# Autodesk Inventor assembly: Trunk
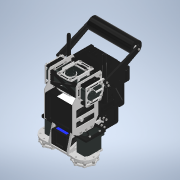
[picture p0: Inventor's stored thumbnail of the model, 180x180]
Saved by Autodesk Inventor 2020.4 (Build 244396000, 396)
## iProperties
Created: 2021-09-10
Part Number: Trunk
Document SubType Name: Assembly
Designer: Masato
Mass: 1663.74 g
Surface Area: 5902.56 cm^2
Volume: 962.647 cm^3
Density: 1.72829 g/cm^3
Author: Masato
## Documents named in this file (38)
- C:\Users\Masato\Documents\Inventor\CIT Brains_Inventor\OpenPlatform_ver3_0\UpperBody\Trunk\Trunk.iam
- C:\Users\Masato\Documents\Inventor\CIT Brains_Inventor\OpenPlatform_ver3_0\UpperBody\Trunk\Trunk_horizontal_frame_03.ipt
- C:\Users\Masato\Documents\Inventor\CIT Brains_Inventor\OpenPlatform_ver3_0\UpperBody\Trunk\Trunk_horizontal_frame_04.ipt
- C:\Users\Masato\Documents\Inventor\CIT Brains_Inventor\OpenPlatform_ver3_0\UpperBody\Trunk\Trunk_horizontal_frame_05.ipt
- C:\Users\Masato\Documents\Inventor\CIT Brains_Inventor\OpenPlatform_ver3_0\UpperBody\Trunk\Trunk_vertical_frame_02.ipt
- C:\Users\Masato\Documents\Inventor\CIT Brains_Inventor\OpenPlatform_ver3_0\UpperBody\Trunk\Trunk_vertical_frame_03.ipt
- C:\Users\Masato\Documents\Inventor\CIT Brains_Inventor\OpenPlatform_ver3_0\UpperBody\Trunk\Trunk_vertical_frame_04.ipt
- C:\Users\Masato\Documents\Inventor\CIT Brains_Inventor\OpenPlatform_ver3_0\UpperBody\Trunk\Trunk_vertical_frame_05.ipt
- C:\Users\Masato\Documents\Inventor\CIT Brains_Inventor\OpenPlatform_ver3_0\UpperBody\Trunk\Trunk_vertical_frame_06.ipt
- C:\Users\Masato\Documents\Inventor\CIT Brains_Inventor\OpenPlatform_ver3_0\Ready_Made\B3M11xx.ipt
- C:\Users\Masato\Documents\Inventor\CIT Brains_Inventor\OpenPlatform_ver3_0\Ready_Made\S3-07-3W.ipt
- C:\Users\Masato\Documents\Inventor\CIT Brains_Inventor\OpenPlatform_ver3_0\Ready_Made\ASU-375H.ipt
- C:\Users\Masato\Documents\Inventor\CIT Brains_Inventor\OpenPlatform_ver3_0\Ready_Made\MSU-306-03.ipt
- C:\Users\Masato\Documents\Inventor\CIT Brains_Inventor\OpenPlatform_ver3_0\Ready_Made\SLSBF7-130-M3-N3.ipt
- C:\Users\Masato\Documents\Inventor\CIT Brains_Inventor\OpenPlatform_ver3_0\Ready_Made\B3M10xx.ipt
- C:\Users\Masato\Documents\Inventor\CIT Brains_Inventor\OpenPlatform_ver3_0\Ready_Made\SGB-100.ipt
- C:\Users\Masato\Documents\Inventor\CIT Brains_Inventor\OpenPlatform_ver3_0\UpperBody\Cockpit\Cockpit.iam
- C:\Users\Masato\Documents\Inventor\CIT Brains_Inventor\OpenPlatform_ver3_0\UpperBody\Trunk\Trunk_vertical_frame_04_MIR.ipt
- C:\Users\Masato\Documents\Inventor\CIT Brains_Inventor\OpenPlatform_ver3_0\UpperBody\Trunk\Trunk_vertical_frame_01.ipt
- C:\Users\Masato\Documents\Inventor\CIT Brains_Inventor\OpenPlatform_ver3_0\UpperBody\Trunk\Trunk_vertical_frame_01_MIR.ipt
- C:\Users\Masato\Documents\Inventor\CIT Brains_Inventor\OpenPlatform_ver3_0\Ready_Made\Screw\SPNFL-BRN-M3-6.ipt
- C:\Users\Masato\Documents\Inventor\CIT Brains_Inventor\OpenPlatform_ver3_0\Ready_Made\Screw\M2_6-15.ipt
- C:\Users\Masato\Documents\Inventor\CIT Brains_Inventor\OpenPlatform_ver3_0\Ready_Made\Screw\M3-8.ipt
- C:\Users\Masato\Documents\Inventor\CIT Brains_Inventor\OpenPlatform_ver3_0\Ready_Made\Screw\M3-6.ipt
- C:\Users\Masato\Documents\Inventor\CIT Brains_Inventor\OpenPlatform_ver3_0\Ready_Made\Screw\M2_6-20.ipt
- C:\Users\Masato\Documents\Inventor\CIT Brains_Inventor\OpenPlatform_ver3_0\UpperBody\Trunk\Outer_support_stand.ipt
- C:\Users\Masato\Documents\Inventor\CIT Brains_Inventor\OpenPlatform_ver3_0\Ready_Made\BRU-307S.ipt
- C:\Users\Masato\Documents\Inventor\CIT Brains_Inventor\OpenPlatform_ver3_0\UpperBody\Trunk\Outer_flange.ipt
- C:\Users\Masato\Documents\Inventor\CIT Brains_Inventor\OpenPlatform_ver3_0\UpperBody\Trunk\Inner_flange.ipt
- C:\Users\Masato\Documents\Inventor\CIT Brains_Inventor\OpenPlatform_ver3_0\Ready_Made\CRBA02508WWC8P5\CRBA02508WWC8P5.ipt
- C:\Users\Masato\Documents\Inventor\CIT Brains_Inventor\OpenPlatform_ver3_0\UpperBody\Trunk\Inner_support_stand.ipt
- C:\Users\Masato\Documents\Inventor\CIT Brains_Inventor\OpenPlatform_ver3_0\UpperBody\Trunk\Trunk_horizontal_frame_01.ipt
- C:\Users\Masato\Documents\Inventor\CIT Brains_Inventor\OpenPlatform_ver3_0\Ready_Made\SF319.ipt
- C:\Users\Masato\Documents\Inventor\CIT Brains_Inventor\OpenPlatform_ver3_0\Ready_Made\BRU-2609S.ipt
- C:\Users\Masato\Documents\Inventor\CIT Brains_Inventor\OpenPlatform_ver3_0\Ready_Made\Screw\M2_6-8.ipt
- C:\Users\Masato\Documents\Inventor\CIT Brains_Inventor\OpenPlatform_ver3_0\UpperBody\Trunk\Trunk_horizontal_frame_02.ipt
- C:\Users\Masato\Documents\Inventor\CIT Brains_Inventor\OpenPlatform_ver3_0\Ready_Made\UUW-0312-10BH.ipt
- C:\Users\Masato\Documents\Inventor\CIT Brains_Inventor\OpenPlatform_ver3_0\Ready_Made\Screw\M2_6-6.ipt
## Components (229 placed, 37 different names)
1. Trunk_horizontal_frame_03:1 — 挿入:172, 挿入:173, 挿入:174, 挿入:175, 挿入:177, 挿入:179, 挿入:255, 挿入:256, 挿入:261, 挿入:262, 挿入:347, 挿入:348, 挿入:463, 挿入:464
2. Trunk_horizontal_frame_03:2 — 挿入:181, 挿入:182, 挿入:184, 挿入:185, 挿入:186, 挿入:187, 挿入:257, 挿入:258, 挿入:337, 挿入:338, 挿入:465, 挿入:466
3. Trunk_horizontal_frame_04:1 — 挿入:115, 挿入:116, 挿入:117, 挿入:118, 挿入:172, 挿入:173, 挿入:181, 挿入:182
4. Trunk_horizontal_frame_04:2 — 挿入:154, 挿入:155, 挿入:156, 挿入:157, 挿入:174, 挿入:175, 挿入:185, 挿入:187
5. Trunk_horizontal_frame_05:1 — 挿入:111, 挿入:112, 挿入:126, 挿入:127
6. Trunk_horizontal_frame_05:2 — 挿入:162, 挿入:163, 挿入:164, 挿入:165
7. Trunk_horizontal_frame_05:3 — 挿入:229, 挿入:230, 挿入:231, 挿入:232
8. Trunk_horizontal_frame_05:4 — 挿入:166, 挿入:167, 挿入:168, 挿入:169
9. Trunk_vertical_frame_01:1 — 角度:35, 角度:36, 挿入:200, 挿入:201, 挿入:420, 挿入:421, 挿入:426, 挿入:501, 挿入:502
10. Trunk_vertical_frame_01_MIR:1 — 角度:37, 角度:38, 挿入:202, 挿入:203, メイト:23, メイト:24, メイト:25, 挿入:418, 挿入:419, 挿入:499, 挿入:500
11. Trunk_vertical_frame_02:1 — フラッシュ:16, メイト:17, フラッシュ:18, フラッシュ:20, フラッシュ:21, メイト:22
12. Trunk_vertical_frame_02:2 — フラッシュ:16, メイト:17, フラッシュ:18, メイト:19
13. Trunk_vertical_frame_02:3 — フラッシュ:15, メイト:18, フラッシュ:17, フラッシュ:19, フラッシュ:20, フラッシュ:21, メイト:21, メイト:20
14. Trunk_vertical_frame_02:4 — フラッシュ:15, メイト:18, フラッシュ:17, メイト:25
15. Trunk_vertical_frame_03:1 — 挿入:101, 挿入:102, 挿入:103, 挿入:111, 挿入:112, 挿入:115, 挿入:116, 挿入:156, 挿入:157, 挿入:164, 挿入:165, フラッシュ:19, メイト:21, 挿入:208, 挿入:226, 挿入:245, 挿入:246, 挿入:247, 挿入:251, 挿入:252, 挿入:327, 挿入:328, 挿入:329, 挿入:330, 挿入:349, 挿入:350
16. Trunk_vertical_frame_03:2 — 挿入:104, 挿入:105, 挿入:106, 挿入:117, 挿入:118, 挿入:154, 挿入:155, 挿入:168, 挿入:169, メイト:22, 挿入:227, 挿入:229, 挿入:230, 挿入:248, 挿入:249, 挿入:250, 挿入:253, 挿入:254, 挿入:331, 挿入:332, 挿入:333, 挿入:334, 挿入:351, 挿入:352
17. Trunk_vertical_frame_04:1 — 挿入:142, 挿入:143, 挿入:144, 挿入:145, 角度:31, 角度:32, 挿入:150, 挿入:151, 挿入:166, 挿入:167, 挿入:231, 挿入:232, 挿入:315, 挿入:316, 挿入:317, 挿入:318, 挿入:323, 挿入:324, 挿入:325, 挿入:326
18. Trunk_vertical_frame_04_MIR:1 — 挿入:124, 挿入:125, 挿入:126, 挿入:127, 挿入:128, 挿入:129, 挿入:136, 挿入:137, 角度:33, 角度:34, 挿入:152, 挿入:153, 挿入:162, 挿入:163, 挿入:311, 挿入:312, 挿入:313, 挿入:314, 挿入:319, 挿入:320, 挿入:321, 挿入:322
19. Trunk_vertical_frame_05:1 — 角度:17, 角度:18, 挿入:75, 挿入:76, 角度:21, 挿入:79, メイト:16, 挿入:263, 挿入:264, 挿入:267
20. Trunk_vertical_frame_05:2 — 角度:19, 挿入:77, 挿入:78, 角度:20, 角度:22, 挿入:80, 挿入:265, 挿入:266, 挿入:268
21. Trunk_vertical_frame_06:1 — 挿入:467, 挿入:468, 挿入:469, 挿入:470, 挿入:471, 挿入:472, 挿入:473, 挿入:474
22. Trunk_vertical_frame_06:2 — 挿入:475, 挿入:476, 挿入:477, 挿入:478, 挿入:479, 挿入:480, 挿入:481, 挿入:482
23. B3M11xx:1 — 角度:39, 挿入:391, 挿入:392, 挿入:422, 挿入:423, 挿入:424, 挿入:425, 挿入:483, 挿入:486
24. B3M11xx:2 — 挿入:427, 挿入:428, 挿入:429, 挿入:484, 挿入:485, 挿入:529
25. B3M11xx:3 — 挿入:177, 挿入:179, 挿入:184, 挿入:186
26. B3M10xx:4 — 挿入:124, 挿入:125, 挿入:128, 挿入:129, 挿入:475, 挿入:476, 挿入:477, 挿入:478
27. B3M10xx:5 — 挿入:142, 挿入:143, 挿入:144, 挿入:145, 挿入:467, 挿入:468, 挿入:469, 挿入:470
28. S3-07-3W:1 — 角度:37, 挿入:202
29. S3-07-3W:2 — 角度:38, 挿入:203
30. S3-07-3W:3 — 角度:36, 挿入:201
31. S3-07-3W:4 — 角度:35, 挿入:200
32. S3-07-3W:5 — 角度:33, 挿入:152
33. S3-07-3W:6 — 角度:34, 挿入:153
34. S3-07-3W:7 — 角度:31, 挿入:150
35. S3-07-3W:8 — 角度:32, 挿入:151
36. ASU-375H:1 — フラッシュ:9, フラッシュ:10, フラッシュ:11, フラッシュ:12, 挿入:101, 挿入:104, メイト:19, メイト:20, メイト:23, メイト:24
37. ASU-375H:2 — フラッシュ:9, フラッシュ:11, 挿入:102, 挿入:105
38. ASU-375H:3 — フラッシュ:10, フラッシュ:12, 挿入:103, 挿入:106
39. MSU-306-03:5 — 角度:17, 挿入:75, 挿入:136
40. MSU-306-03:6 — 角度:18, 挿入:76, 挿入:137
41. MSU-306-03:11 — 角度:19, 挿入:77
42. MSU-306-03:12 — 挿入:78, 角度:20
43. SLSBF7-130-M3-N3:1 — 角度:21, 角度:22, 挿入:79, 挿入:80, メイト:15
44. SGB-100:1 — メイト:15, メイト:16
45. Cockpit:1 [sub-assembly] — 挿入:208, 角度:39
46. SPNFL-BRN-M3-6:1 — 挿入:226
47. SPNFL-BRN-M3-6:2 — 挿入:227
48. M3-8:5 — 挿入:245
49. M3-8:6 — 挿入:246
50. M3-8:7 — 挿入:247
51. M3-8:8 — 挿入:248
52. M3-8:9 — 挿入:249
53. M3-8:10 — 挿入:250
54. M3-6:1 — 挿入:251
55. M3-6:2 — 挿入:252
56. M3-6:3 — 挿入:254
57. M3-6:4 — 挿入:253
58. M3-6:5 — 挿入:256
59. M3-6:6 — 挿入:255
60. M3-6:7 — 挿入:258
61. M3-6:8 — 挿入:257
62. M2_6-15:9 — 挿入:464
63. M2_6-15:10 — 挿入:463
64. M2_6-15:11 — 挿入:261
65. M2_6-15:12 — 挿入:262
66. M3-6:9 — 挿入:263
67. M3-6:10 — 挿入:264
68. M3-6:11 — 挿入:266
69. M3-6:12 — 挿入:265
70. M3-8:11 — 挿入:267
71. M3-8:12 — 挿入:268
72. M2_6-20:1 — 挿入:489
73. M2_6-20:2 — 挿入:490
74. M2_6-20:3 — 挿入:487
75. M2_6-20:4 — 挿入:488
76. M2_6-15:13 — 挿入:311
77. M2_6-15:14 — 挿入:312
78. M2_6-15:15 — 挿入:313
79. M2_6-15:16 — 挿入:314
80. M2_6-15:17 — 挿入:315
81. M2_6-15:18 — 挿入:316
82. M2_6-15:19 — 挿入:317
83. M2_6-15:20 — 挿入:318
84. M3-6:13 — 挿入:319
85. M3-6:14 — 挿入:320
86. M3-6:15 — 挿入:321
87. M3-6:16 — 挿入:322
88. M3-6:17 — 挿入:323
89. M3-6:18 — 挿入:324
90. M3-6:19 — 挿入:325
91. M3-6:20 — 挿入:326
92. M3-6:21 — 挿入:327
93. M3-6:22 — 挿入:328
94. M3-6:23 — 挿入:329
95. M3-6:24 — 挿入:330
96. M3-6:25 — 挿入:331
97. M3-6:26 — 挿入:332
98. M3-6:27 — 挿入:333
99. M3-6:28 — 挿入:334
100. M2_6-20:9 — 挿入:465
101. M2_6-20:10 — 挿入:466
102. M2_6-20:11 — 挿入:337
103. M2_6-20:12 — 挿入:338
104. M2_6-20:13 — 挿入:479
105. M2_6-20:14 — 挿入:482
106. M2_6-20:15 — 挿入:481
107. M2_6-20:16 — 挿入:480
108. M2_6-20:17 — 挿入:474
109. M2_6-20:18 — 挿入:472
110. M2_6-20:19 — 挿入:473
111. M2_6-20:20 — 挿入:471
112. M3-6:29 — 挿入:347
113. M3-6:30 — 挿入:348
114. M3-6:31 — 挿入:349
115. M3-6:32 — 挿入:350
116. M3-6:33 — 挿入:351
117. M3-6:34 — 挿入:352
118. Outer_support_stand:1 — 挿入:371, 挿入:372, 挿入:373, 挿入:374, 挿入:375, 挿入:376, 挿入:377, 挿入:378, 挿入:397, 挿入:438, 挿入:439
119. BRU-307S:1 — 挿入:371, 挿入:404
120. BRU-307S:2 — 挿入:372
121. BRU-307S:3 — 挿入:373
122. BRU-307S:4 — 挿入:374
123. BRU-307S:5 — 挿入:375, 挿入:405
124. BRU-307S:6 — 挿入:376
125. BRU-307S:7 — 挿入:377
126. BRU-307S:8 — 挿入:378
127. Inner_flange:1 — 挿入:391, 挿入:392, 挿入:452, 挿入:453, 挿入:454, 挿入:455
128. CRBA02508WWC8P5:1 — 挿入:397
129. Inner_support_stand:1 — 角度:40, 挿入:398, 角度:41, 挿入:399, 角度:42, 挿入:400, 角度:43, 挿入:401, 挿入:456, 挿入:457, 挿入:458, 挿入:459, 挿入:460, 挿入:461
130. S3-07-3W:9 — 角度:40, 挿入:398
131. S3-07-3W:10 — 角度:41, 挿入:399
132. S3-07-3W:11 — 角度:42, 挿入:400
133. S3-07-3W:12 — 角度:43, 挿入:401
134. Outer_flange:1 — 挿入:404, 挿入:405, 挿入:406, 挿入:407, 挿入:408, 挿入:409, 挿入:410, 挿入:411, 挿入:412, 挿入:413
135. M3-6:35 — 挿入:406
136. M3-6:36 — 挿入:407
137. M3-6:37 — 挿入:408
138. M3-6:38 — 挿入:409
139. M3-6:39 — 挿入:410
140. M3-6:40 — 挿入:411
141. M3-6:41 — 挿入:412
142. M3-6:42 — 挿入:413
143. Trunk_horizontal_frame_01:1 — 挿入:418, 挿入:419, 挿入:420, 挿入:421, 挿入:422, 挿入:423, 挿入:424, 挿入:425, 挿入:426, 挿入:427, 挿入:428, 挿入:429, 挿入:430, 挿入:431, 挿入:432, 挿入:433, 挿入:434, 挿入:435, 挿入:436, 挿入:440, 挿入:441, 挿入:442, 挿入:443, 挿入:444, 挿入:445, 挿入:446, 挿入:447, 挿入:448, 挿入:449, 挿入:450, 挿入:451, フラッシュ:22, 挿入:462, 挿入:511, 挿入:512, 挿入:513, 挿入:514, 挿入:515, 挿入:516, 挿入:517, 挿入:518
144. SF319:1 — 挿入:430
145. SF319:2 — 挿入:431
146. SF319:3 — 挿入:432
147. SF319:4 — 挿入:433, 挿入:439
148. SF319:5 — 挿入:434
149. SF319:6 — 挿入:435
150. SF319:7 — 挿入:436, 挿入:438
151. SF319:8 — 挿入:462
152. M2_6-15:21 — 挿入:441
153. M2_6-15:22 — 挿入:440
154. M2_6-15:23 — 挿入:442
155. M2_6-15:24 — 挿入:443
156. M2_6-15:25 — 挿入:444
157. M2_6-15:26 — 挿入:445
158. M2_6-15:27 — 挿入:446
159. M2_6-15:28 — 挿入:447
160. M3-8:13 — 挿入:448
161. M3-8:14 — 挿入:449
162. M3-8:15 — 挿入:450
163. M3-8:16 — 挿入:451
164. BRU-2609S:1 — 挿入:455, 挿入:457
165. BRU-2609S:2 — 挿入:454
166. BRU-2609S:3 — 挿入:453
167. BRU-2609S:4 — 挿入:452, 挿入:456
168. M2_6-8:1 — 挿入:458
169. M2_6-8:2 — 挿入:459
170. M2_6-8:3 — 挿入:460
171. M2_6-8:4 — 挿入:461
172. Trunk_horizontal_frame_02:1 — 挿入:483, 挿入:484, 挿入:485, 挿入:486, 挿入:487, 挿入:488, 挿入:489, 挿入:490
173. BRU-307S:9 — 挿入:497, 挿入:503
174. BRU-307S:10 — 挿入:498, 挿入:504
175. BRU-307S:11 — 挿入:496, 挿入:506
176. BRU-307S:12 — 挿入:495, 挿入:505
177. UUW-0312-10BH:1 — 挿入:495, 挿入:507
178. UUW-0312-10BH:2 — 挿入:496, 挿入:508
179. UUW-0312-10BH:3 — 挿入:497, 挿入:509
180. UUW-0312-10BH:4 — 挿入:498, 挿入:510
181. UUW-0312-10BH:5 — 挿入:499, 挿入:505
182. UUW-0312-10BH:6 — 挿入:500, 挿入:506
183. UUW-0312-10BH:7 — 挿入:501, 挿入:503
184. UUW-0312-10BH:8 — 挿入:502, 挿入:504
185. M3-6:43 — 挿入:507
186. M3-6:44 — 挿入:508
187. M3-6:45 — 挿入:510
188. M3-6:46 — 挿入:509
189. SF319:9 — 挿入:511, 挿入:519
190. SF319:10 — 挿入:512
191. SF319:11 — 挿入:513
192. SF319:12 — 挿入:514
193. SF319:13 — 挿入:515, 挿入:520
194. SF319:14 — 挿入:516
195. SF319:15 — 挿入:517
196. SF319:16 — 挿入:518
197. Outer_support_stand:2 — 挿入:519, 挿入:520, 挿入:521, 挿入:522, 挿入:523, 挿入:524, 挿入:525, 挿入:526, 挿入:527, 挿入:528, 挿入:554
198. BRU-307S:13 — 挿入:521, 挿入:534
199. BRU-307S:14 — 挿入:522
200. BRU-307S:15 — 挿入:523
201. BRU-307S:16 — 挿入:524
202. BRU-307S:17 — 挿入:525, 挿入:535
203. BRU-307S:18 — 挿入:526
204. BRU-307S:19 — 挿入:527
205. BRU-307S:20 — 挿入:528
206. BRU-2609S:5 — 挿入:530, 挿入:540
207. BRU-2609S:6 — 挿入:531, 挿入:541
208. BRU-2609S:7 — 挿入:532
209. BRU-2609S:8 — 挿入:533
210. S3-07-3W:13 — 角度:44, 挿入:536
211. S3-07-3W:14 — 角度:45, 挿入:537
212. S3-07-3W:15 — 角度:46, 挿入:538
213. S3-07-3W:16 — 角度:47, 挿入:539
214. Inner_flange:2 — 挿入:529, 挿入:530, 挿入:531, 挿入:532, 挿入:533
215. Inner_support_stand:2 — 角度:44, 挿入:536, 角度:45, 挿入:537, 角度:46, 挿入:538, 角度:47, 挿入:539, 挿入:540, 挿入:541, 挿入:550, 挿入:551, 挿入:552, 挿入:553
216. Outer_flange:2 — 挿入:534, 挿入:535, 挿入:542, 挿入:543, 挿入:544, 挿入:545, 挿入:546, 挿入:547, 挿入:548, 挿入:549
217. M3-6:47 — 挿入:542
218. M3-6:48 — 挿入:543
219. M3-6:49 — 挿入:544
220. M3-6:50 — 挿入:545
221. M3-6:51 — 挿入:546
222. M3-6:52 — 挿入:547
223. M3-6:53 — 挿入:548
224. M3-6:54 — 挿入:549
225. M2_6-6:1 — 挿入:550
226. M2_6-6:2 — 挿入:551
227. M2_6-6:3 — 挿入:552
228. M2_6-6:4 — 挿入:553
229. CRBA02508WWC8P5:2 — 挿入:554
## Relationships (326: Insert 280, Angle 23, Flush 12, Mate 11)
- フラッシュ:9 [Flush]: ASU-375H:1 ↔ ASU-375H:2
- フラッシュ:10 [Flush]: ASU-375H:1 ↔ ASU-375H:3
- フラッシュ:11 [Flush]: ASU-375H:1 ↔ ASU-375H:2
- フラッシュ:12 [Flush]: ASU-375H:1 ↔ ASU-375H:3
- 角度:17 [Angle] (0 deg): Trunk_vertical_frame_05:1 ↔ MSU-306-03:5
- 角度:18 [Angle] (0 deg): Trunk_vertical_frame_05:1 ↔ MSU-306-03:6
- 挿入:75 [Insert]: Trunk_vertical_frame_05:1 ↔ MSU-306-03:5
- 挿入:76 [Insert]: Trunk_vertical_frame_05:1 ↔ MSU-306-03:6
- 角度:19 [Angle] (0 deg): Trunk_vertical_frame_05:2 ↔ MSU-306-03:11
- 挿入:77 [Insert]: Trunk_vertical_frame_05:2 ↔ MSU-306-03:11
- 挿入:78 [Insert]: Trunk_vertical_frame_05:2 ↔ MSU-306-03:12
- 角度:20 [Angle] (0 deg): Trunk_vertical_frame_05:2 ↔ MSU-306-03:12
- 角度:21 [Angle] (0 deg): Trunk_vertical_frame_05:1 ↔ SLSBF7-130-M3-N3:1
- 角度:22 [Angle] (0 deg): Trunk_vertical_frame_05:2 ↔ SLSBF7-130-M3-N3:1
- 挿入:79 [Insert]: Trunk_vertical_frame_05:1 ↔ SLSBF7-130-M3-N3:1
- 挿入:80 [Insert]: Trunk_vertical_frame_05:2 ↔ SLSBF7-130-M3-N3:1
- メイト:15 [Mate]: SLSBF7-130-M3-N3:1 ↔ SGB-100:1
- メイト:16 [Mate] (2.5 mm): Trunk_vertical_frame_05:1 ↔ SGB-100:1
- 挿入:101 [Insert]: Trunk_vertical_frame_03:1 ↔ ASU-375H:1
- 挿入:102 [Insert]: Trunk_vertical_frame_03:1 ↔ ASU-375H:2
- 挿入:103 [Insert]: Trunk_vertical_frame_03:1 ↔ ASU-375H:3
- 挿入:104 [Insert]: Trunk_vertical_frame_03:2 ↔ ASU-375H:1
- 挿入:105 [Insert]: Trunk_vertical_frame_03:2 ↔ ASU-375H:2
- 挿入:106 [Insert]: Trunk_vertical_frame_03:2 ↔ ASU-375H:3
- 挿入:111 [Insert]: Trunk_horizontal_frame_05:1 ↔ Trunk_vertical_frame_03:1
- 挿入:112 [Insert]: Trunk_horizontal_frame_05:1 ↔ Trunk_vertical_frame_03:1
- 挿入:115 [Insert]: Trunk_horizontal_frame_04:1 ↔ Trunk_vertical_frame_03:1
- 挿入:116 [Insert]: Trunk_horizontal_frame_04:1 ↔ Trunk_vertical_frame_03:1
- 挿入:117 [Insert]: Trunk_horizontal_frame_04:1 ↔ Trunk_vertical_frame_03:2
- 挿入:118 [Insert]: Trunk_horizontal_frame_04:1 ↔ Trunk_vertical_frame_03:2
- 挿入:124 [Insert]: Trunk_vertical_frame_04_MIR:1 ↔ B3M10xx:4
- 挿入:125 [Insert]: Trunk_vertical_frame_04_MIR:1 ↔ B3M10xx:4
- 挿入:126 [Insert]: Trunk_horizontal_frame_05:1 ↔ Trunk_vertical_frame_04_MIR:1
- 挿入:127 [Insert]: Trunk_horizontal_frame_05:1 ↔ Trunk_vertical_frame_04_MIR:1
- 挿入:128 [Insert]: Trunk_vertical_frame_04_MIR:1 ↔ B3M10xx:4
- 挿入:129 [Insert]: Trunk_vertical_frame_04_MIR:1 ↔ B3M10xx:4
- 挿入:136 [Insert]: Trunk_vertical_frame_04_MIR:1 ↔ MSU-306-03:5
- 挿入:137 [Insert]: Trunk_vertical_frame_04_MIR:1 ↔ MSU-306-03:6
- 挿入:142 [Insert]: Trunk_vertical_frame_04:1 ↔ B3M10xx:5
- 挿入:143 [Insert]: Trunk_vertical_frame_04:1 ↔ B3M10xx:5
- 挿入:144 [Insert]: Trunk_vertical_frame_04:1 ↔ B3M10xx:5
- 挿入:145 [Insert]: Trunk_vertical_frame_04:1 ↔ B3M10xx:5
- 角度:31 [Angle] (0 deg): Trunk_vertical_frame_04:1 ↔ S3-07-3W:7
- 角度:32 [Angle] (0 deg): Trunk_vertical_frame_04:1 ↔ S3-07-3W:8
- 挿入:150 [Insert]: Trunk_vertical_frame_04:1 ↔ S3-07-3W:7
- 挿入:151 [Insert]: Trunk_vertical_frame_04:1 ↔ S3-07-3W:8
- 角度:33 [Angle] (0 deg): Trunk_vertical_frame_04_MIR:1 ↔ S3-07-3W:5
- 角度:34 [Angle] (0 deg): Trunk_vertical_frame_04_MIR:1 ↔ S3-07-3W:6
- 挿入:152 [Insert]: Trunk_vertical_frame_04_MIR:1 ↔ S3-07-3W:5
- 挿入:153 [Insert]: Trunk_vertical_frame_04_MIR:1 ↔ S3-07-3W:6
- 挿入:154 [Insert]: Trunk_horizontal_frame_04:2 ↔ Trunk_vertical_frame_03:2
- 挿入:155 [Insert]: Trunk_horizontal_frame_04:2 ↔ Trunk_vertical_frame_03:2
- 挿入:156 [Insert]: Trunk_horizontal_frame_04:2 ↔ Trunk_vertical_frame_03:1
- 挿入:157 [Insert]: Trunk_horizontal_frame_04:2 ↔ Trunk_vertical_frame_03:1
- 挿入:162 [Insert]: Trunk_horizontal_frame_05:2 ↔ Trunk_vertical_frame_04_MIR:1
- 挿入:163 [Insert]: Trunk_horizontal_frame_05:2 ↔ Trunk_vertical_frame_04_MIR:1
- 挿入:164 [Insert]: Trunk_horizontal_frame_05:2 ↔ Trunk_vertical_frame_03:1
- 挿入:165 [Insert]: Trunk_horizontal_frame_05:2 ↔ Trunk_vertical_frame_03:1
- 挿入:166 [Insert]: Trunk_horizontal_frame_05:4 ↔ Trunk_vertical_frame_04:1
- 挿入:167 [Insert]: Trunk_horizontal_frame_05:4 ↔ Trunk_vertical_frame_04:1
- 挿入:168 [Insert]: Trunk_horizontal_frame_05:4 ↔ Trunk_vertical_frame_03:2
- 挿入:169 [Insert]: Trunk_horizontal_frame_05:4 ↔ Trunk_vertical_frame_03:2
- 挿入:172 [Insert]: Trunk_horizontal_frame_03:1 ↔ Trunk_horizontal_frame_04:1
- 挿入:173 [Insert]: Trunk_horizontal_frame_03:1 ↔ Trunk_horizontal_frame_04:1
- 挿入:174 [Insert]: Trunk_horizontal_frame_03:1 ↔ Trunk_horizontal_frame_04:2
- 挿入:175 [Insert]: Trunk_horizontal_frame_03:1 ↔ Trunk_horizontal_frame_04:2
- 挿入:177 [Insert]: Trunk_horizontal_frame_03:1 ↔ B3M11xx:3
- 挿入:179 [Insert]: Trunk_horizontal_frame_03:1 ↔ B3M11xx:3
- 挿入:181 [Insert]: Trunk_horizontal_frame_03:2 ↔ Trunk_horizontal_frame_04:1
- 挿入:182 [Insert]: Trunk_horizontal_frame_03:2 ↔ Trunk_horizontal_frame_04:1
- 挿入:184 [Insert]: Trunk_horizontal_frame_03:2 ↔ B3M11xx:3
- 挿入:185 [Insert]: Trunk_horizontal_frame_03:2 ↔ Trunk_horizontal_frame_04:2
- 挿入:186 [Insert]: Trunk_horizontal_frame_03:2 ↔ B3M11xx:3
- 挿入:187 [Insert]: Trunk_horizontal_frame_03:2 ↔ Trunk_horizontal_frame_04:2
- フラッシュ:15 [Flush]: Trunk_vertical_frame_02:3 ↔ Trunk_vertical_frame_02:4
- フラッシュ:16 [Flush]: Trunk_vertical_frame_02:1 ↔ Trunk_vertical_frame_02:2
- メイト:17 [Mate]: Trunk_vertical_frame_02:1 ↔ Trunk_vertical_frame_02:2
- メイト:18 [Mate]: Trunk_vertical_frame_02:3 ↔ Trunk_vertical_frame_02:4
- フラッシュ:17 [Flush]: Trunk_vertical_frame_02:3 ↔ Trunk_vertical_frame_02:4
- フラッシュ:18 [Flush]: Trunk_vertical_frame_02:1 ↔ Trunk_vertical_frame_02:2
- フラッシュ:19 [Flush]: Trunk_vertical_frame_02:3 ↔ Trunk_vertical_frame_03:1
- フラッシュ:20 [Flush]: Trunk_vertical_frame_02:1 ↔ Trunk_vertical_frame_02:3
- メイト:19 [Mate] (0.01 mm): Trunk_vertical_frame_02:2 ↔ ASU-375H:1
- メイト:20 [Mate] (0.01 mm): Trunk_vertical_frame_02:3 ↔ ASU-375H:1
- フラッシュ:21 [Flush]: Trunk_vertical_frame_02:1 ↔ Trunk_vertical_frame_02:3
- メイト:21 [Mate]: Trunk_vertical_frame_02:3 ↔ Trunk_vertical_frame_03:1
- メイト:22 [Mate]: Trunk_vertical_frame_02:1 ↔ Trunk_vertical_frame_03:2
- 角度:35 [Angle] (0 deg): Trunk_vertical_frame_01:1 ↔ S3-07-3W:4
- 角度:36 [Angle] (0 deg): Trunk_vertical_frame_01:1 ↔ S3-07-3W:3
- 挿入:200 [Insert]: Trunk_vertical_frame_01:1 ↔ S3-07-3W:4
- 挿入:201 [Insert]: Trunk_vertical_frame_01:1 ↔ S3-07-3W:3
- 角度:37 [Angle] (0 deg): Trunk_vertical_frame_01_MIR:1 ↔ S3-07-3W:1
- 角度:38 [Angle] (0 deg): Trunk_vertical_frame_01_MIR:1 ↔ S3-07-3W:2
- 挿入:202 [Insert]: Trunk_vertical_frame_01_MIR:1 ↔ S3-07-3W:1
- 挿入:203 [Insert]: Trunk_vertical_frame_01_MIR:1 ↔ S3-07-3W:2
- メイト:23 [Mate] (0.01 mm): Trunk_vertical_frame_01_MIR:1 ↔ ASU-375H:1
- メイト:24 [Mate] (0.01 mm): Trunk_vertical_frame_01_MIR:1 ↔ ASU-375H:1
- メイト:25 [Mate]: Trunk_vertical_frame_01_MIR:1 ↔ Trunk_vertical_frame_02:4
- 挿入:208 [Insert] (0.25 mm): Trunk_vertical_frame_03:1 ↔ Cockpit:1
- 角度:39 [Angle] (0 deg): B3M11xx:1 ↔ Cockpit:1
- 挿入:226 [Insert]: Trunk_vertical_frame_03:1 ↔ SPNFL-BRN-M3-6:1
- 挿入:227 [Insert]: Trunk_vertical_frame_03:2 ↔ SPNFL-BRN-M3-6:2
- 挿入:229 [Insert]: Trunk_horizontal_frame_05:3 ↔ Trunk_vertical_frame_03:2
- 挿入:230 [Insert]: Trunk_horizontal_frame_05:3 ↔ Trunk_vertical_frame_03:2
- 挿入:231 [Insert]: Trunk_horizontal_frame_05:3 ↔ Trunk_vertical_frame_04:1
- 挿入:232 [Insert]: Trunk_horizontal_frame_05:3 ↔ Trunk_vertical_frame_04:1
- 挿入:245 [Insert]: Trunk_vertical_frame_03:1 ↔ M3-8:5
- 挿入:246 [Insert]: Trunk_vertical_frame_03:1 ↔ M3-8:6
- 挿入:247 [Insert]: Trunk_vertical_frame_03:1 ↔ M3-8:7
- 挿入:248 [Insert]: Trunk_vertical_frame_03:2 ↔ M3-8:8
- 挿入:249 [Insert]: Trunk_vertical_frame_03:2 ↔ M3-8:9
- 挿入:250 [Insert]: Trunk_vertical_frame_03:2 ↔ M3-8:10
- 挿入:251 [Insert]: Trunk_vertical_frame_03:1 ↔ M3-6:1
- 挿入:252 [Insert]: Trunk_vertical_frame_03:1 ↔ M3-6:2
- 挿入:253 [Insert]: Trunk_vertical_frame_03:2 ↔ M3-6:4
- 挿入:254 [Insert]: Trunk_vertical_frame_03:2 ↔ M3-6:3
- 挿入:255 [Insert]: Trunk_horizontal_frame_03:1 ↔ M3-6:6
- 挿入:256 [Insert]: Trunk_horizontal_frame_03:1 ↔ M3-6:5
- 挿入:257 [Insert]: Trunk_horizontal_frame_03:2 ↔ M3-6:8
- 挿入:258 [Insert]: Trunk_horizontal_frame_03:2 ↔ M3-6:7
- 挿入:261 [Insert]: Trunk_horizontal_frame_03:1 ↔ M2_6-15:11
- 挿入:262 [Insert]: Trunk_horizontal_frame_03:1 ↔ M2_6-15:12
- 挿入:263 [Insert]: Trunk_vertical_frame_05:1 ↔ M3-6:9
- 挿入:264 [Insert]: Trunk_vertical_frame_05:1 ↔ M3-6:10
- 挿入:265 [Insert]: Trunk_vertical_frame_05:2 ↔ M3-6:12
- 挿入:266 [Insert]: Trunk_vertical_frame_05:2 ↔ M3-6:11
- 挿入:267 [Insert]: Trunk_vertical_frame_05:1 ↔ M3-8:11
- 挿入:268 [Insert]: Trunk_vertical_frame_05:2 ↔ M3-8:12
- 挿入:311 [Insert]: Trunk_vertical_frame_04_MIR:1 ↔ M2_6-15:13
- 挿入:312 [Insert]: Trunk_vertical_frame_04_MIR:1 ↔ M2_6-15:14
- 挿入:313 [Insert]: Trunk_vertical_frame_04_MIR:1 ↔ M2_6-15:15
- 挿入:314 [Insert]: Trunk_vertical_frame_04_MIR:1 ↔ M2_6-15:16
- 挿入:315 [Insert]: Trunk_vertical_frame_04:1 ↔ M2_6-15:17
- 挿入:316 [Insert]: Trunk_vertical_frame_04:1 ↔ M2_6-15:18
- 挿入:317 [Insert]: Trunk_vertical_frame_04:1 ↔ M2_6-15:19
- 挿入:318 [Insert]: Trunk_vertical_frame_04:1 ↔ M2_6-15:20
- 挿入:319 [Insert]: Trunk_vertical_frame_04_MIR:1 ↔ M3-6:13
- 挿入:320 [Insert]: Trunk_vertical_frame_04_MIR:1 ↔ M3-6:14
- 挿入:321 [Insert]: Trunk_vertical_frame_04_MIR:1 ↔ M3-6:15
- 挿入:322 [Insert]: Trunk_vertical_frame_04_MIR:1 ↔ M3-6:16
- 挿入:323 [Insert]: Trunk_vertical_frame_04:1 ↔ M3-6:17
- 挿入:324 [Insert]: Trunk_vertical_frame_04:1 ↔ M3-6:18
- 挿入:325 [Insert]: Trunk_vertical_frame_04:1 ↔ M3-6:19
- 挿入:326 [Insert]: Trunk_vertical_frame_04:1 ↔ M3-6:20
- 挿入:327 [Insert]: Trunk_vertical_frame_03:1 ↔ M3-6:21
- 挿入:328 [Insert]: Trunk_vertical_frame_03:1 ↔ M3-6:22
- 挿入:329 [Insert]: Trunk_vertical_frame_03:1 ↔ M3-6:23
- 挿入:330 [Insert]: Trunk_vertical_frame_03:1 ↔ M3-6:24
- 挿入:331 [Insert]: Trunk_vertical_frame_03:2 ↔ M3-6:25
- 挿入:332 [Insert]: Trunk_vertical_frame_03:2 ↔ M3-6:26
- 挿入:333 [Insert]: Trunk_vertical_frame_03:2 ↔ M3-6:27
- 挿入:334 [Insert]: Trunk_vertical_frame_03:2 ↔ M3-6:28
- 挿入:337 [Insert]: Trunk_horizontal_frame_03:2 ↔ M2_6-20:11
- 挿入:338 [Insert]: Trunk_horizontal_frame_03:2 ↔ M2_6-20:12
- 挿入:347 [Insert]: Trunk_horizontal_frame_03:1 ↔ M3-6:29
- 挿入:348 [Insert]: Trunk_horizontal_frame_03:1 ↔ M3-6:30
- 挿入:349 [Insert]: Trunk_vertical_frame_03:1 ↔ M3-6:31
- 挿入:350 [Insert]: Trunk_vertical_frame_03:1 ↔ M3-6:32
- 挿入:351 [Insert]: Trunk_vertical_frame_03:2 ↔ M3-6:33
- 挿入:352 [Insert]: Trunk_vertical_frame_03:2 ↔ M3-6:34
- 挿入:371 [Insert]: Outer_support_stand:1 ↔ BRU-307S:1
- 挿入:372 [Insert]: Outer_support_stand:1 ↔ BRU-307S:2
- 挿入:373 [Insert]: Outer_support_stand:1 ↔ BRU-307S:3
- 挿入:374 [Insert]: Outer_support_stand:1 ↔ BRU-307S:4
- 挿入:375 [Insert]: Outer_support_stand:1 ↔ BRU-307S:5
- 挿入:376 [Insert]: Outer_support_stand:1 ↔ BRU-307S:6
- 挿入:377 [Insert]: Outer_support_stand:1 ↔ BRU-307S:7
- 挿入:378 [Insert]: Outer_support_stand:1 ↔ BRU-307S:8
- 挿入:391 [Insert]: B3M11xx:1 ↔ Inner_flange:1
- 挿入:392 [Insert]: B3M11xx:1 ↔ Inner_flange:1
- 挿入:397 [Insert]: Outer_support_stand:1 ↔ CRBA02508WWC8P5:1
- 角度:40 [Angle] (0 deg): Inner_support_stand:1 ↔ S3-07-3W:9
- 挿入:398 [Insert]: Inner_support_stand:1 ↔ S3-07-3W:9
- 角度:41 [Angle] (0 deg): Inner_support_stand:1 ↔ S3-07-3W:10
- 挿入:399 [Insert]: Inner_support_stand:1 ↔ S3-07-3W:10
- 角度:42 [Angle] (0 deg): Inner_support_stand:1 ↔ S3-07-3W:11
- 挿入:400 [Insert]: Inner_support_stand:1 ↔ S3-07-3W:11
- 角度:43 [Angle] (0 deg): Inner_support_stand:1 ↔ S3-07-3W:12
- 挿入:401 [Insert]: Inner_support_stand:1 ↔ S3-07-3W:12
- 挿入:404 [Insert]: BRU-307S:1 ↔ Outer_flange:1
- 挿入:405 [Insert]: BRU-307S:5 ↔ Outer_flange:1
- 挿入:406 [Insert]: Outer_flange:1 ↔ M3-6:35
- 挿入:407 [Insert]: Outer_flange:1 ↔ M3-6:36
- 挿入:408 [Insert]: Outer_flange:1 ↔ M3-6:37
- 挿入:409 [Insert]: Outer_flange:1 ↔ M3-6:38
- 挿入:410 [Insert]: Outer_flange:1 ↔ M3-6:39
- 挿入:411 [Insert]: Outer_flange:1 ↔ M3-6:40
- 挿入:412 [Insert]: Outer_flange:1 ↔ M3-6:41
- 挿入:413 [Insert]: Outer_flange:1 ↔ M3-6:42
- 挿入:418 [Insert]: Trunk_vertical_frame_01_MIR:1 ↔ Trunk_horizontal_frame_01:1
- 挿入:419 [Insert]: Trunk_vertical_frame_01_MIR:1 ↔ Trunk_horizontal_frame_01:1
- 挿入:420 [Insert]: Trunk_vertical_frame_01:1 ↔ Trunk_horizontal_frame_01:1
- 挿入:421 [Insert]: Trunk_vertical_frame_01:1 ↔ Trunk_horizontal_frame_01:1
- 挿入:422 [Insert]: B3M11xx:1 ↔ Trunk_horizontal_frame_01:1
- 挿入:423 [Insert]: B3M11xx:1 ↔ Trunk_horizontal_frame_01:1
- 挿入:424 [Insert]: B3M11xx:1 ↔ Trunk_horizontal_frame_01:1
- 挿入:425 [Insert]: B3M11xx:1 ↔ Trunk_horizontal_frame_01:1
- 挿入:426 [Insert]: Trunk_vertical_frame_01:1 ↔ Trunk_horizontal_frame_01:1
- 挿入:427 [Insert]: B3M11xx:2 ↔ Trunk_horizontal_frame_01:1
- 挿入:428 [Insert]: B3M11xx:2 ↔ Trunk_horizontal_frame_01:1
- 挿入:429 [Insert]: B3M11xx:2 ↔ Trunk_horizontal_frame_01:1
- 挿入:430 [Insert]: Trunk_horizontal_frame_01:1 ↔ SF319:1
- 挿入:431 [Insert]: Trunk_horizontal_frame_01:1 ↔ SF319:2
- 挿入:432 [Insert]: Trunk_horizontal_frame_01:1 ↔ SF319:3
- 挿入:433 [Insert]: Trunk_horizontal_frame_01:1 ↔ SF319:4
- 挿入:434 [Insert]: Trunk_horizontal_frame_01:1 ↔ SF319:5
- 挿入:435 [Insert]: Trunk_horizontal_frame_01:1 ↔ SF319:6
- 挿入:436 [Insert]: Trunk_horizontal_frame_01:1 ↔ SF319:7
- 挿入:438 [Insert]: Outer_support_stand:1 ↔ SF319:7
- 挿入:439 [Insert]: Outer_support_stand:1 ↔ SF319:4
- 挿入:440 [Insert]: Trunk_horizontal_frame_01:1 ↔ M2_6-15:22
- 挿入:441 [Insert]: Trunk_horizontal_frame_01:1 ↔ M2_6-15:21
- 挿入:442 [Insert]: Trunk_horizontal_frame_01:1 ↔ M2_6-15:23
- 挿入:443 [Insert]: Trunk_horizontal_frame_01:1 ↔ M2_6-15:24
- 挿入:444 [Insert]: Trunk_horizontal_frame_01:1 ↔ M2_6-15:25
- 挿入:445 [Insert]: Trunk_horizontal_frame_01:1 ↔ M2_6-15:26
- 挿入:446 [Insert]: Trunk_horizontal_frame_01:1 ↔ M2_6-15:27
- 挿入:447 [Insert]: Trunk_horizontal_frame_01:1 ↔ M2_6-15:28
- 挿入:448 [Insert]: Trunk_horizontal_frame_01:1 ↔ M3-8:13
- 挿入:449 [Insert]: Trunk_horizontal_frame_01:1 ↔ M3-8:14
- 挿入:450 [Insert]: Trunk_horizontal_frame_01:1 ↔ M3-8:15
- 挿入:451 [Insert]: Trunk_horizontal_frame_01:1 ↔ M3-8:16
- 挿入:452 [Insert]: Inner_flange:1 ↔ BRU-2609S:4
- 挿入:453 [Insert]: Inner_flange:1 ↔ BRU-2609S:3
- 挿入:454 [Insert]: Inner_flange:1 ↔ BRU-2609S:2
- 挿入:455 [Insert]: Inner_flange:1 ↔ BRU-2609S:1
- 挿入:456 [Insert]: Inner_support_stand:1 ↔ BRU-2609S:4
- 挿入:457 [Insert]: Inner_support_stand:1 ↔ BRU-2609S:1
- 挿入:458 [Insert]: Inner_support_stand:1 ↔ M2_6-8:1
- 挿入:459 [Insert]: Inner_support_stand:1 ↔ M2_6-8:2
- 挿入:460 [Insert]: Inner_support_stand:1 ↔ M2_6-8:3
- 挿入:461 [Insert]: Inner_support_stand:1 ↔ M2_6-8:4
- フラッシュ:22 [Flush]: Trunk_horizontal_frame_01:1
- 挿入:462 [Insert]: Trunk_horizontal_frame_01:1 ↔ SF319:8
- 挿入:463 [Insert]: Trunk_horizontal_frame_03:1 ↔ M2_6-15:10
- 挿入:464 [Insert]: Trunk_horizontal_frame_03:1 ↔ M2_6-15:9
- 挿入:465 [Insert]: Trunk_horizontal_frame_03:2 ↔ M2_6-20:9
- 挿入:466 [Insert]: Trunk_horizontal_frame_03:2 ↔ M2_6-20:10
- 挿入:467 [Insert]: Trunk_vertical_frame_06:1 ↔ B3M10xx:5
- 挿入:468 [Insert]: Trunk_vertical_frame_06:1 ↔ B3M10xx:5
- 挿入:469 [Insert]: Trunk_vertical_frame_06:1 ↔ B3M10xx:5
- 挿入:470 [Insert]: Trunk_vertical_frame_06:1 ↔ B3M10xx:5
- 挿入:471 [Insert]: Trunk_vertical_frame_06:1 ↔ M2_6-20:20
- 挿入:472 [Insert]: Trunk_vertical_frame_06:1 ↔ M2_6-20:18
- 挿入:473 [Insert]: Trunk_vertical_frame_06:1 ↔ M2_6-20:19
- 挿入:474 [Insert]: Trunk_vertical_frame_06:1 ↔ M2_6-20:17
- 挿入:475 [Insert]: Trunk_vertical_frame_06:2 ↔ B3M10xx:4
- 挿入:476 [Insert]: Trunk_vertical_frame_06:2 ↔ B3M10xx:4
- 挿入:477 [Insert]: Trunk_vertical_frame_06:2 ↔ B3M10xx:4
- 挿入:478 [Insert]: Trunk_vertical_frame_06:2 ↔ B3M10xx:4
- 挿入:479 [Insert]: Trunk_vertical_frame_06:2 ↔ M2_6-20:13
- 挿入:480 [Insert]: Trunk_vertical_frame_06:2 ↔ M2_6-20:16
- 挿入:481 [Insert]: Trunk_vertical_frame_06:2 ↔ M2_6-20:15
- 挿入:482 [Insert]: Trunk_vertical_frame_06:2 ↔ M2_6-20:14
- 挿入:483 [Insert]: B3M11xx:1 ↔ Trunk_horizontal_frame_02:1
- 挿入:484 [Insert]: B3M11xx:2 ↔ Trunk_horizontal_frame_02:1
- 挿入:485 [Insert]: B3M11xx:2 ↔ Trunk_horizontal_frame_02:1
- 挿入:486 [Insert]: B3M11xx:1 ↔ Trunk_horizontal_frame_02:1
- 挿入:487 [Insert]: M2_6-20:3 ↔ Trunk_horizontal_frame_02:1
- 挿入:488 [Insert]: M2_6-20:4 ↔ Trunk_horizontal_frame_02:1
- 挿入:489 [Insert]: M2_6-20:1 ↔ Trunk_horizontal_frame_02:1
- 挿入:490 [Insert]: M2_6-20:2 ↔ Trunk_horizontal_frame_02:1
- 挿入:495 [Insert]: BRU-307S:12 ↔ UUW-0312-10BH:1
- 挿入:496 [Insert]: BRU-307S:11 ↔ UUW-0312-10BH:2
- 挿入:497 [Insert]: BRU-307S:9 ↔ UUW-0312-10BH:3
- 挿入:498 [Insert]: BRU-307S:10 ↔ UUW-0312-10BH:4
- 挿入:499 [Insert]: Trunk_vertical_frame_01_MIR:1 ↔ UUW-0312-10BH:5
- 挿入:500 [Insert]: Trunk_vertical_frame_01_MIR:1 ↔ UUW-0312-10BH:6
- 挿入:501 [Insert]: Trunk_vertical_frame_01:1 ↔ UUW-0312-10BH:7
- 挿入:502 [Insert]: Trunk_vertical_frame_01:1 ↔ UUW-0312-10BH:8
- 挿入:503 [Insert]: BRU-307S:9 ↔ UUW-0312-10BH:7
- 挿入:504 [Insert]: BRU-307S:10 ↔ UUW-0312-10BH:8
- 挿入:505 [Insert]: BRU-307S:12 ↔ UUW-0312-10BH:5
- 挿入:506 [Insert]: BRU-307S:11 ↔ UUW-0312-10BH:6
- 挿入:507 [Insert]: UUW-0312-10BH:1 ↔ M3-6:43
- 挿入:508 [Insert]: UUW-0312-10BH:2 ↔ M3-6:44
- 挿入:509 [Insert]: UUW-0312-10BH:3 ↔ M3-6:46
- 挿入:510 [Insert]: UUW-0312-10BH:4 ↔ M3-6:45
- 挿入:511 [Insert]: Trunk_horizontal_frame_01:1 ↔ SF319:9
- 挿入:512 [Insert]: Trunk_horizontal_frame_01:1 ↔ SF319:10
- 挿入:513 [Insert]: Trunk_horizontal_frame_01:1 ↔ SF319:11
- 挿入:514 [Insert]: Trunk_horizontal_frame_01:1 ↔ SF319:12
- 挿入:515 [Insert]: Trunk_horizontal_frame_01:1 ↔ SF319:13
- 挿入:516 [Insert]: Trunk_horizontal_frame_01:1 ↔ SF319:14
- 挿入:517 [Insert]: Trunk_horizontal_frame_01:1 ↔ SF319:15
- 挿入:518 [Insert]: Trunk_horizontal_frame_01:1 ↔ SF319:16
- 挿入:519 [Insert]: SF319:9 ↔ Outer_support_stand:2
- 挿入:520 [Insert]: SF319:13 ↔ Outer_support_stand:2
- 挿入:521 [Insert]: Outer_support_stand:2 ↔ BRU-307S:13
- 挿入:522 [Insert]: Outer_support_stand:2 ↔ BRU-307S:14
- 挿入:523 [Insert]: Outer_support_stand:2 ↔ BRU-307S:15
- 挿入:524 [Insert]: Outer_support_stand:2 ↔ BRU-307S:16
- 挿入:525 [Insert]: Outer_support_stand:2 ↔ BRU-307S:17
- 挿入:526 [Insert]: Outer_support_stand:2 ↔ BRU-307S:18
- 挿入:527 [Insert]: Outer_support_stand:2 ↔ BRU-307S:19
- 挿入:528 [Insert]: Outer_support_stand:2 ↔ BRU-307S:20
- 挿入:529 [Insert]: B3M11xx:2 ↔ Inner_flange:2
- 挿入:530 [Insert]: BRU-2609S:5 ↔ Inner_flange:2
- 挿入:531 [Insert]: BRU-2609S:6 ↔ Inner_flange:2
- 挿入:532 [Insert]: BRU-2609S:7 ↔ Inner_flange:2
- 挿入:533 [Insert]: BRU-2609S:8 ↔ Inner_flange:2
- 挿入:534 [Insert]: BRU-307S:13 ↔ Outer_flange:2
- 挿入:535 [Insert]: BRU-307S:17 ↔ Outer_flange:2
- 角度:44 [Angle] (0 deg): S3-07-3W:13 ↔ Inner_support_stand:2
- 挿入:536 [Insert]: S3-07-3W:13 ↔ Inner_support_stand:2
- 角度:45 [Angle] (0 deg): S3-07-3W:14 ↔ Inner_support_stand:2
- 挿入:537 [Insert]: S3-07-3W:14 ↔ Inner_support_stand:2
- 角度:46 [Angle] (0 deg): S3-07-3W:15 ↔ Inner_support_stand:2
- 挿入:538 [Insert]: S3-07-3W:15 ↔ Inner_support_stand:2
- 角度:47 [Angle] (0 deg): S3-07-3W:16 ↔ Inner_support_stand:2
- 挿入:539 [Insert]: S3-07-3W:16 ↔ Inner_support_stand:2
- 挿入:540 [Insert]: BRU-2609S:5 ↔ Inner_support_stand:2
- 挿入:541 [Insert]: BRU-2609S:6 ↔ Inner_support_stand:2
- 挿入:542 [Insert]: Outer_flange:2 ↔ M3-6:47
- 挿入:543 [Insert]: Outer_flange:2 ↔ M3-6:48
- 挿入:544 [Insert]: Outer_flange:2 ↔ M3-6:49
- 挿入:545 [Insert]: Outer_flange:2 ↔ M3-6:50
- 挿入:546 [Insert]: Outer_flange:2 ↔ M3-6:51
- 挿入:547 [Insert]: Outer_flange:2 ↔ M3-6:52
- 挿入:548 [Insert]: Outer_flange:2 ↔ M3-6:53
- 挿入:549 [Insert]: Outer_flange:2 ↔ M3-6:54
- 挿入:550 [Insert]: Inner_support_stand:2 ↔ M2_6-6:1
- 挿入:551 [Insert]: Inner_support_stand:2 ↔ M2_6-6:2
- 挿入:552 [Insert]: Inner_support_stand:2 ↔ M2_6-6:3
- 挿入:553 [Insert]: Inner_support_stand:2 ↔ M2_6-6:4
- 挿入:554 [Insert]: Outer_support_stand:2 ↔ CRBA02508WWC8P5:2
